# Autodesk Inventor assembly: !Create 3 Public Model
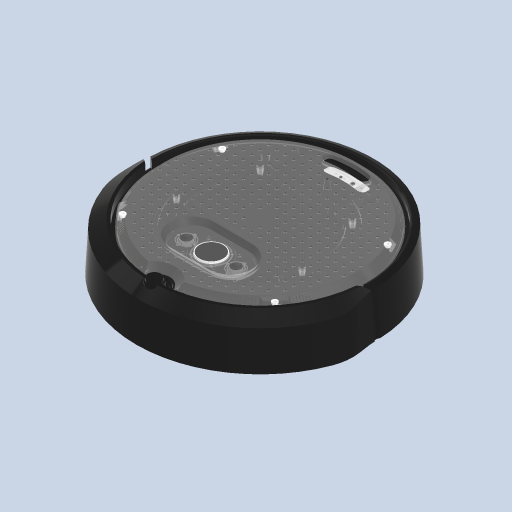
[picture p0: Inventor's stored thumbnail of the model, 512x512]
Saved by Autodesk Inventor 2024 (Build 280153000, 153)
## iProperties
Company: iRobot Corporation
Created: 2022-01-19
Part Number: !Create 3 Public Model
Description: Model of iRobot Create 3 robot.
Document SubType Name: Assembly
Designer: Greg
Sending System: Autodesk Translation Framework v10.10.0.1391
Preprocessor: ST-DEVELOPER v18.1
Title: Create 3 Model 20220119.step
Author: Raphael Cherney
## Documents named in this file (5)
- C:\Users\Greg\Documents\Inventor\Capstone\iRobot_Create_3_Public_Model\iRobot_Create_3_Public_Model.iam
- C:\Users\Greg\Documents\Inventor\Capstone\iRobot_Create_3_Public_Model\Simplified Body.ipt
- C:\Users\Greg\Documents\Inventor\Capstone\iRobot_Create_3_Public_Model\Faceplate Assembly.iam
- C:\Users\Greg\Documents\Inventor\Capstone\iRobot_Create_3_Public_Model\Locating Pins.iam
- C:\Users\Greg\Documents\Inventor\Capstone\iRobot_Create_3_Public_Model\Cargo Bay Assembly.iam
## Components (4 placed, 4 different names)
1. Simplified Body:1 — Mate:1, Mate:3, Mate:4, Mate:5, Mate:6, Flush:1, Mate:7
2. Faceplate Assembly:1 [sub-assembly] — Mate:1, Mate:2, Mate:6
3. Locating Pins:1 [sub-assembly] — Mate:2, Mate:3, Mate:4, Mate:5
4. Cargo Bay Assembly:1 [sub-assembly] — Flush:1, Mate:7
## Relationships (8: Mate 7, Flush 1)
- Mate:1: Simplified Body:1 ↔ Faceplate Assembly:1
- Mate:2: Faceplate Assembly:1 ↔ Locating Pins:1
- Mate:3: Simplified Body:1 ↔ Locating Pins:1
- Mate:4: Simplified Body:1 ↔ Locating Pins:1
- Mate:5: Simplified Body:1 ↔ Locating Pins:1
- Mate:6: Simplified Body:1 ↔ Faceplate Assembly:1
- Flush:1: Simplified Body:1 ↔ Cargo Bay Assembly:1
- Mate:7: Simplified Body:1 ↔ Cargo Bay Assembly:1
